# Autodesk Inventor assembly: PCB Stack
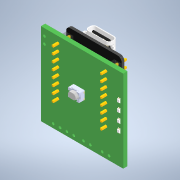
[picture p0: Inventor's stored thumbnail of the model, 180x180]
Saved by Autodesk Inventor 2022 (Build 260153000, 153)
## iProperties
Created: 2023-11-16
Part Number: PCB Stack
Document SubType Name: Assembly
Designer: mbrzo
Author: mbrzo
## Documents named in this file (5)
- C:\Users\mbrzo\Documents\ALRT_v1\PCB Stack.iam
- C:\Users\mbrzo\Documents\ALRT_v1\ALRT_v1.iam
- C:\Users\mbrzo\Documents\ALRT_v1\beetle ESP32-C3.iam
- C:\Users\mbrzo\Documents\ALRT_v1\PTS810 SJM 250 SMTR LFS--3DModel-STEP-56544.ipt
- C:\Users\mbrzo\Documents\ALRT_v1\LTST-C191KGKT--3DModel-STEP-56544.ipt
## Components (7 placed, 4 different names)
1. ALRT_v1:1 [sub-assembly] — Mate:1, Mate:2, Mate:3, Mate:4, Mate:5, Mate:6, Mate:7, Mate:8, Mate:9, Mate:10, Mate:11, Mate:12
2. beetle ESP32-C3:1 [sub-assembly] — Mate:1
3. PTS810 SJM 250 SMTR LFS--3DModel-STEP-56544:1 — Mate:2, Mate:3, Mate:4
4. LTST-C191KGKT--3DModel-STEP-56544:1 — Mate:5, Mate:6, Mate:7
5. LTST-C191KGKT--3DModel-STEP-56544:2 — Mate:8, Mate:9, Mate:10
6. LTST-C191KGKT--3DModel-STEP-56544:3 — Mate:11
7. LTST-C191KGKT--3DModel-STEP-56544:4 — Mate:12
## Relationships (12: Mate 12)
- Mate:1: ALRT_v1:1 ↔ beetle ESP32-C3:1
- Mate:2: ALRT_v1:1 ↔ PTS810 SJM 250 SMTR LFS--3DModel-STEP-56544:1
- Mate:3 (14.25 mm): ALRT_v1:1 ↔ PTS810 SJM 250 SMTR LFS--3DModel-STEP-56544:1
- Mate:4 (12.45 mm): ALRT_v1:1 ↔ PTS810 SJM 250 SMTR LFS--3DModel-STEP-56544:1
- Mate:5: ALRT_v1:1 ↔ LTST-C191KGKT--3DModel-STEP-56544:1
- Mate:6 (-1.8 mm): ALRT_v1:1 ↔ LTST-C191KGKT--3DModel-STEP-56544:1
- Mate:7 (-10 mm): ALRT_v1:1 ↔ LTST-C191KGKT--3DModel-STEP-56544:1
- Mate:8: ALRT_v1:1 ↔ LTST-C191KGKT--3DModel-STEP-56544:2
- Mate:9 (1 mm): ALRT_v1:1 ↔ LTST-C191KGKT--3DModel-STEP-56544:2
- Mate:10 (10.75 mm): ALRT_v1:1 ↔ LTST-C191KGKT--3DModel-STEP-56544:2
- Mate:11: ALRT_v1:1 ↔ LTST-C191KGKT--3DModel-STEP-56544:3
- Mate:12: ALRT_v1:1 ↔ LTST-C191KGKT--3DModel-STEP-56544:4
